# Autodesk Inventor assembly: Panel Mount Vertical Support for 4040 - Assembly
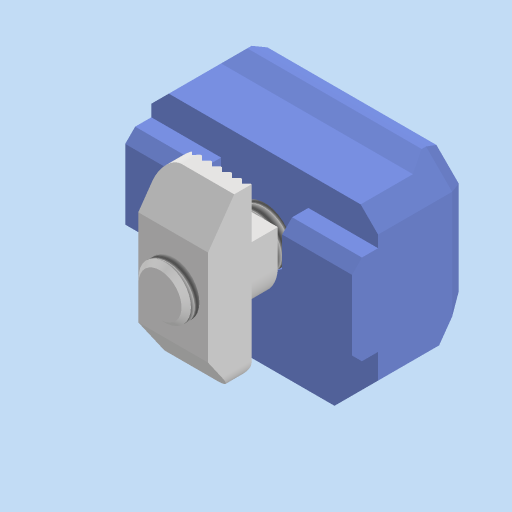
[picture p0: Inventor's stored thumbnail of the model, 512x512]
Saved by Autodesk Inventor 2023.2 (Build 272271000, 271)
## iProperties
Created: 2023-12-04
Part Number: Panel Mount Vertical Support for 4040 - Assembly
Document SubType Name: Assembly
Designer: Nils Bade
Author: Nils Bade
## Documents named in this file (4)
- C:\Users\nilsb\Documents\Inventor\Projektarbeit-Bade\Enclosure\Panel Mount Vertical Support for 4040 - Assembly.iam
- C:\Users\nilsb\Documents\Inventor\Projektarbeit-Bade\Enclosure\Panel Mount Vertical Support for 4040.ipt
- C:\Users\nilsb\Documents\Inventor\Projektarbeit-Bade\RatRig_modified\T-NUT - DropIn 4040 SERIES - M6.ipt
- C:\Users\nilsb\Documents\Inventor\Projektarbeit-Bade\Schrauben\Cap Head Screw M6x16 - DIN912.ipt
## Components (3 placed, 3 different names)
1. T-NUT - DROP IN TYPE FOR 40 SERIES - M6:1
2. Cap Head Screw M6x16 - DIN912:1
3. Panel Mount Vertical Support for 4040:1
## Relationships (5: Mate 4, Angle 1)
- [Mate]: T-NUT - DROP IN TYPE FOR 40 SERIES - M6:1 ↔ Panel Mount Vertical Support for 4040:1
- [Angle] (0 deg): T-NUT - DROP IN TYPE FOR 40 SERIES - M6:1 ↔ Panel Mount Vertical Support for 4040:1
- [Mate] (5.5 mm): T-NUT - DROP IN TYPE FOR 40 SERIES - M6:1 ↔ Panel Mount Vertical Support for 4040:1
- [Mate]: Cap Head Screw M6x16 - DIN912:1 ↔ Panel Mount Vertical Support for 4040:1
- [Mate]: Cap Head Screw M6x16 - DIN912:1 ↔ Panel Mount Vertical Support for 4040:1
